# Autodesk Inventor assembly: GŁÓWKA CIĘGŁA SI 05 TK
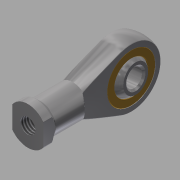
[picture p0: Inventor's stored thumbnail of the model, 180x180]
Saved by Autodesk Inventor 2013 (Build 170138000, 138)
## iProperties
Created: 2015-04-17
Part Number: GŁÓWKA CIĘGŁA SI 05 TK
Document SubType Name: Assembly
Designer: Ultimate
Author: Ultimate
## Documents named in this file (4)
- C:\Users\Ultimate\Desktop\STRATO3D\STÓŁ GRZEWCZY\GŁÓWKA CIĘGŁA SI 05 TK\GŁÓWKA CIĘGŁA SI 05 TK.iam
- C:\Users\Ultimate\Desktop\STRATO3D\STÓŁ GRZEWCZY\GŁÓWKA CIĘGŁA SI 05 TK\KORPUS.ipt
- C:\Users\Ultimate\Desktop\STRATO3D\STÓŁ GRZEWCZY\GŁÓWKA CIĘGŁA SI 05 TK\KULA.ipt
- C:\Users\Ultimate\Desktop\STRATO3D\STÓŁ GRZEWCZY\GŁÓWKA CIĘGŁA SI 05 TK\TULEJA.ipt
## Components (3 placed, 3 different names)
1. KORPUS:1 — Flush:1, Mate:1
2. KULA:1 — Tangent:1
3. TULEJA:1 — Flush:1, Mate:1, Tangent:1
## Relationships (3: Flush 1, Mate 1, Tangent 1)
- Flush:1: KORPUS:1 ↔ TULEJA:1
- Mate:1: KORPUS:1 ↔ TULEJA:1
- Tangent:1: KULA:1 ↔ TULEJA:1
